# Autodesk Inventor assembly: LensMount
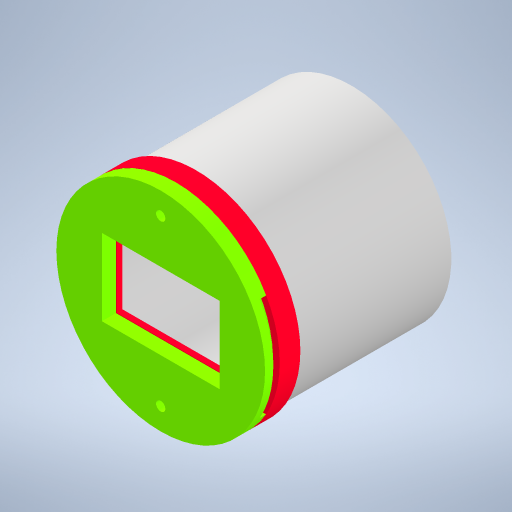
[picture p0: Inventor's stored thumbnail of the model, 512x512]
Saved by Autodesk Inventor 2023 (Build 270158000, 158)
## iProperties
Created: 2022-10-31
Part Number: LensMount
Document SubType Name: Assembly
Designer: Piotr
Author: Piotr
## Documents named in this file (4)
- H:\3d\FilmScanner\LensMount.iam
- H:\3d\FilmScanner\LensMount_mount.ipt
- H:\3d\FilmScanner\LensMount_frame.ipt
- H:\3d\FilmScanner\FilmGuide.ipt
## Components (3 placed, 3 different names)
1. LensMount_mount:1 — Flush:1
2. LensMount_frame:1 — Flush:1, Flush:2
3. FilmGuide:1 — Flush:2
## Relationships (2: Flush 2)
- Flush:1: LensMount_mount:1 ↔ LensMount_frame:1
- Flush:2: LensMount_frame:1 ↔ FilmGuide:1
